# Autodesk Inventor assembly: Assembly
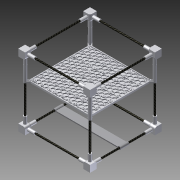
[picture p0: Inventor's stored thumbnail of the model, 180x180]
Saved by Autodesk Inventor 2011 (Build 150239000, 239)
## iProperties
Created: 2011-07-20
Part Number: Assembly
Document SubType Name: Assembly
Designer: Seb Madgwick
Author: Seb Madgwick
## Documents named in this file (5)
- C:\MyFiles\x-io\Products\x-IMU Calibration Cube\x-IMU Calibration Cube Mechanical\x-IMU Calibration Cube.iam
- C:\MyFiles\x-io\Products\x-IMU Calibration Cube\x-IMU Calibration Cube Mechanical\x-IMU Calibration Cube Stage.ipt
- C:\MyFiles\x-io\Products\x-IMU Calibration Cube\x-IMU Calibration Cube Mechanical\x-IMU Calibration Cube Rod.ipt
- C:\MyFiles\x-io\Products\x-IMU Calibration Cube\x-IMU Calibration Cube Mechanical\x-IMU Calibration Cube Corner.ipt
- C:\MyFiles\x-io\Products\x-IMU Calibration Cube\x-IMU Calibration Cube Mechanical\x-IMU Calibration Cube Bracket.ipt
## Components (22 placed, 5 different names)
1. x-IMU Calibration Cube Stage:1 — Mate:1, Mate:2, Mate:3, Mate:4, Mate:5
2. x-IMU Calibration Cube Corner:1 — Insert:1, Insert:2, Insert:22
3. x-IMU Calibration Cube Corner:2 — Insert:3, Insert:4, Insert:7
4. x-IMU Calibration Cube Corner:3 — Insert:5, Insert:6
5. x-IMU Calibration Cube Corner:4 — Insert:8, Insert:9, Insert:10
6. x-IMU Calibration Cube Corner:6 — Insert:13, Insert:14, Insert:21, Mate:5
7. x-IMU Calibration Cube Corner:5 — Insert:11, Insert:12, Insert:17
8. x-IMU Calibration Cube Corner:7 — Insert:15, Insert:16
9. x-IMU Calibration Cube Corner:8 — Insert:18, Insert:19, Insert:20
10. x-IMU Calibration Cube Rod:1 — Mate:4, Insert:3, Insert:11
11. x-IMU Calibration Cube Rod:2 — Mate:3, Insert:1, Insert:14
12. x-IMU Calibration Cube Rod:3 — Mate:2, Insert:8, Insert:18
13. x-IMU Calibration Cube Rod:4 — Mate:1, Insert:5, Insert:15
14. x-IMU Calibration Cube Rod:5 — Insert:2, Insert:4, Mate:7
15. x-IMU Calibration Cube Rod:6 — Insert:6, Insert:7
16. x-IMU Calibration Cube Rod:7 — Insert:9, Insert:22
17. Rod:8 — Insert:12, Insert:13
18. Rod:9 — Insert:16, Insert:17
19. Rod:10 — Insert:20, Insert:21
20. Rod:11 — Insert:10, Mate:6
21. Rod:12 — Insert:19
22. x-IMU Calibration Cube Bracket:1 — Mate:6, Mate:7
## Relationships (29: Insert 22, Mate 7)
- Mate:1: x-IMU Calibration Cube Stage:1 ↔ x-IMU Calibration Cube Rod:4
- Mate:2: x-IMU Calibration Cube Stage:1 ↔ x-IMU Calibration Cube Rod:3
- Mate:3: x-IMU Calibration Cube Stage:1 ↔ x-IMU Calibration Cube Rod:2
- Mate:4: x-IMU Calibration Cube Stage:1 ↔ x-IMU Calibration Cube Rod:1
- Insert:1: x-IMU Calibration Cube Corner:1 ↔ x-IMU Calibration Cube Rod:2
- Insert:2: x-IMU Calibration Cube Corner:1 ↔ x-IMU Calibration Cube Rod:5
- Insert:3: x-IMU Calibration Cube Corner:2 ↔ x-IMU Calibration Cube Rod:1
- Insert:4: x-IMU Calibration Cube Corner:2 ↔ x-IMU Calibration Cube Rod:5
- Insert:5: x-IMU Calibration Cube Corner:3 ↔ x-IMU Calibration Cube Rod:4
- Insert:6: x-IMU Calibration Cube Corner:3 ↔ x-IMU Calibration Cube Rod:6
- Insert:7: x-IMU Calibration Cube Corner:2 ↔ x-IMU Calibration Cube Rod:6
- Insert:8: x-IMU Calibration Cube Corner:4 ↔ x-IMU Calibration Cube Rod:3
- Insert:9: x-IMU Calibration Cube Corner:4 ↔ x-IMU Calibration Cube Rod:7
- Insert:10: x-IMU Calibration Cube Corner:4 ↔ Rod:11
- Insert:11: x-IMU Calibration Cube Corner:5 ↔ x-IMU Calibration Cube Rod:1
- Insert:12: x-IMU Calibration Cube Corner:5 ↔ Rod:8
- Insert:13: x-IMU Calibration Cube Corner:6 ↔ Rod:8
- Insert:14: x-IMU Calibration Cube Corner:6 ↔ x-IMU Calibration Cube Rod:2
- Insert:15: x-IMU Calibration Cube Corner:7 ↔ x-IMU Calibration Cube Rod:4
- Insert:16: x-IMU Calibration Cube Corner:7 ↔ Rod:9
- Insert:17: x-IMU Calibration Cube Corner:5 ↔ Rod:9
- Insert:18: x-IMU Calibration Cube Corner:8 ↔ x-IMU Calibration Cube Rod:3
- Insert:19: x-IMU Calibration Cube Corner:8 ↔ Rod:12
- Insert:20: x-IMU Calibration Cube Corner:8 ↔ Rod:10
- Insert:21: x-IMU Calibration Cube Corner:6 ↔ Rod:10
- Insert:22: x-IMU Calibration Cube Corner:1 ↔ x-IMU Calibration Cube Rod:7
- Mate:5: x-IMU Calibration Cube Stage:1 ↔ x-IMU Calibration Cube Corner:6
- Mate:6: Rod:11 ↔ x-IMU Calibration Cube Bracket:1
- Mate:7: x-IMU Calibration Cube Rod:5 ↔ x-IMU Calibration Cube Bracket:1
